# Autodesk Inventor assembly: RightUpperArmUnit
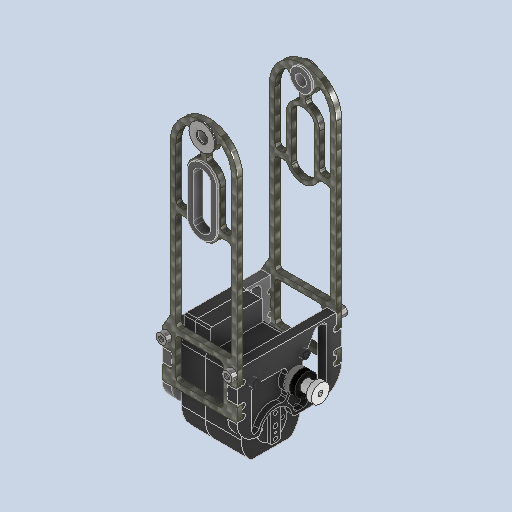
[picture p0: Inventor's stored thumbnail of the model, 512x512]
Saved by Autodesk Inventor 2024.2 (Build 282272000, 272)
## iProperties
Created: 2024-01-18
Part Number: RightUpperArmUnit
Document SubType Name: Assembly
Designer: Masato Kubotera
Mass: 141.771 g
Surface Area: 347.314 cm^2
Volume: 67.2008 cm^3
Density: 2.10967 g/cm^3
Author: Masato Kubotera
## Documents named in this file (16)
- C:\Users\masato\OneDrive - Chiba Institute of Technology\CIT Brains\RoboCup2024\Mechanic\SUSTAINA-OP2-DEV - 作業\NativeFiles\Boby\UpperLimb\UpperArms\RightUpperArmUnit.iam
- C:\Users\masato\OneDrive - Chiba Institute of Technology\CIT Brains\RoboCup2024\Mechanic\SUSTAINA-OP2-DEV - 作業\NativeFiles\Boby\UpperLimb\UpperArms\UpperArmFrame.ipt
- C:\Users\masato\OneDrive - Chiba Institute of Technology\CIT Brains\RoboCup2024\Mechanic\SUSTAINA-OP2-DEV - 作業\NativeFiles\Boby\UpperLimb\UpperArms\UpperArmIdlerSideFrame.ipt
- C:\Users\masato\OneDrive - Chiba Institute of Technology\CIT Brains\RoboCup2024\Mechanic\SUSTAINA-OP2-DEV - 作業\NativeFiles\Boby\COTS\Actuators\PMX-SCR-5203HV.ipt
- C:\Users\masato\OneDrive - Chiba Institute of Technology\CIT Brains\RoboCup2024\Mechanic\SUSTAINA-OP2-DEV - 作業\NativeFiles\Boby\COTS\Screws\CapScrew\UC-0308.ipt
- C:\Users\masato\OneDrive - Chiba Institute of Technology\CIT Brains\RoboCup2024\Mechanic\SUSTAINA-OP2-DEV - 作業\NativeFiles\Boby\COTS\Screws\CapScrew\FC-2615EB.ipt
- C:\Users\masato\OneDrive - Chiba Institute of Technology\CIT Brains\RoboCup2024\Mechanic\SUSTAINA-OP2-DEV - 作業\NativeFiles\Boby\COTS\Washers\Metal\UUW-0614-05H.ipt
- C:\Users\masato\OneDrive - Chiba Institute of Technology\CIT Brains\RoboCup2024\Mechanic\SUSTAINA-OP2-DEV - 作業\NativeFiles\Boby\COTS\Bushes\GFM-0608-04.ipt
- C:\Users\masato\OneDrive - Chiba Institute of Technology\CIT Brains\RoboCup2024\Mechanic\SUSTAINA-OP2-DEV - 作業\NativeFiles\Boby\CommonDesignedComponents\SliderProtectionFrame.ipt
- C:\Users\masato\OneDrive - Chiba Institute of Technology\CIT Brains\RoboCup2024\Mechanic\SUSTAINA-OP2-DEV - 作業\NativeFiles\Boby\COTS\Washers\Resin\CC-0612-30B.ipt
- C:\Users\masato\OneDrive - Chiba Institute of Technology\CIT Brains\RoboCup2024\Mechanic\SUSTAINA-OP2-DEV - 作業\NativeFiles\Boby\COTS\Washers\Metal\UUW-0412-30H.ipt
- C:\Users\masato\OneDrive - Chiba Institute of Technology\CIT Brains\RoboCup2024\Mechanic\SUSTAINA-OP2-DEV - 作業\NativeFiles\Boby\COTS\Washers\Metal\UUW-0412-15H.ipt
- C:\Users\masato\OneDrive - Chiba Institute of Technology\CIT Brains\RoboCup2024\Mechanic\SUSTAINA-OP2-DEV - 作業\NativeFiles\Boby\UpperLimb\UpperArms\UpperArmHornSideFrame_MIR.ipt
- C:\Users\masato\OneDrive - Chiba Institute of Technology\CIT Brains\RoboCup2024\Mechanic\SUSTAINA-OP2-DEV - 作業\NativeFiles\Boby\COTS\Washers\Resin\TT-0614-05.ipt
- C:\Users\masato\OneDrive - Chiba Institute of Technology\CIT Brains\RoboCup2024\Mechanic\SUSTAINA-OP2-DEV - 作業\NativeFiles\Boby\COTS\Screws\ScrewsWithShoulder\DBSY4-5-5.ipt
- C:\Users\masato\OneDrive - Chiba Institute of Technology\CIT Brains\RoboCup2024\Mechanic\SUSTAINA-OP2-DEV - 作業\NativeFiles\Boby\COTS\Screws\ScrewsWithShoulder\DBSY4-8-6.ipt
## Components (23 placed, 15 different names)
1. UpperArmFrame:1 — Mate:1, Angle:1, Insert:7, Insert:13, Insert:19, Insert:21, Insert:25, Insert:35
2. UpperArmIdlerSideFrame:1 — Insert:3, Insert:32, Insert:35
3. UpperArmFrame:2 — Insert:3, Insert:9, Insert:15, Insert:23, Insert:26, Insert:27, Insert:28, Insert:29
4. UpperArmHornSideFrame_MIR:1 — Insert:7, Insert:9, Insert:11, Insert:12, Insert:17, Insert:18, Flush:1, Insert:30
5. SliderProtectionFrame:1 — Insert:27, Insert:28
6. PMX-SCR-5203HV:1 — Insert:11, Insert:12
7. UC-0308:1 — Insert:13
8. UC-0308:3 — Insert:15
9. UC-0308:5 — Insert:19
10. UC-0308:7 — Insert:29
11. FC-2615EB:1 — Insert:17
12. FC-2615EB:2 — Insert:18
13. CC-0612-30B:1 — Insert:31
14. UUW-0412-30H:1 — Insert:30, Insert:31, Insert:34
15. UUW-0412-15H:1 — Insert:32, Insert:33
16. TT-0614-05:2 — Insert:21, Insert:22
17. TT-0614-05:1 — Insert:23, Insert:24
18. UUW-0614-05H:1 — Insert:22
19. UUW-0614-05H:2 — Insert:24
20. GFM-0608-04:1 — Insert:25
21. GFM-0608-04:2 — Insert:26
22. DBSY4-5-5:1 — Insert:33, Mate:2
23. DBSY4-8-6:1 — Insert:34, Mate:2
## Relationships (29: Insert 25, Mate 2, Angle 1, Flush 1)
- Mate:1: UpperArmFrame:1
- Angle:1 (180 deg): UpperArmFrame:1
- Flush:1: UpperArmHornSideFrame_MIR:1
- Insert:3: UpperArmIdlerSideFrame:1 ↔ UpperArmFrame:2
- Insert:7: UpperArmFrame:1 ↔ UpperArmHornSideFrame_MIR:1
- Insert:9: UpperArmFrame:2 ↔ UpperArmHornSideFrame_MIR:1
- Insert:11: UpperArmHornSideFrame_MIR:1 ↔ PMX-SCR-5203HV:1
- Insert:12: UpperArmHornSideFrame_MIR:1 ↔ PMX-SCR-5203HV:1
- Insert:13: UpperArmFrame:1 ↔ UC-0308:1
- Insert:15: UpperArmFrame:2 ↔ UC-0308:3
- Insert:17: UpperArmHornSideFrame_MIR:1 ↔ FC-2615EB:1
- Insert:18: UpperArmHornSideFrame_MIR:1 ↔ FC-2615EB:2
- Insert:19: UpperArmFrame:1 ↔ UC-0308:5
- Insert:21: UpperArmFrame:1 ↔ TT-0614-05:2
- Insert:22: TT-0614-05:2 ↔ UUW-0614-05H:1
- Insert:23: UpperArmFrame:2 ↔ TT-0614-05:1
- Insert:24: TT-0614-05:1 ↔ UUW-0614-05H:2
- Insert:25: UpperArmFrame:1 ↔ GFM-0608-04:1
- Insert:26: UpperArmFrame:2 ↔ GFM-0608-04:2
- Insert:27: UpperArmFrame:2 ↔ SliderProtectionFrame:1
- Insert:28: UpperArmFrame:2 ↔ SliderProtectionFrame:1
- Insert:29: UpperArmFrame:2 ↔ UC-0308:7
- Insert:30: UpperArmHornSideFrame_MIR:1 ↔ UUW-0412-30H:1
- Insert:31: CC-0612-30B:1 ↔ UUW-0412-30H:1
- Insert:32: UpperArmIdlerSideFrame:1 ↔ UUW-0412-15H:1
- Insert:33: UUW-0412-15H:1 ↔ DBSY4-5-5:1
- Insert:34: UUW-0412-30H:1 ↔ DBSY4-8-6:1
- Insert:35: UpperArmFrame:1 ↔ UpperArmIdlerSideFrame:1
- Mate:2: DBSY4-5-5:1 ↔ DBSY4-8-6:1
